# Autodesk Inventor assembly: Assembly1
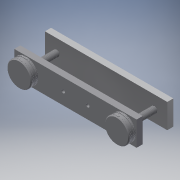
[picture p0: Inventor's stored thumbnail of the model, 180x180]
Saved by Autodesk Inventor 2019 (Build 230136000, 136)
## iProperties
Created: 2019-02-14
Part Number: Assembly1
Document SubType Name: Assembly
Designer: Delta
Author: Delta
## Documents named in this file (4)
- C:\Robotics\2018-19_CAD\lift\Assembly1.iam
- C:\Robotics\2018-19_CAD\Plate that touches lift.ipt
- C:\Robotics\2018-19_CAD\lift\Plate that doewsn't touch lander.ipt
- C:\Robotics\2018-19_CAD\lift\90210A111_LIMITED CLEARANCE SWIVEL-PAD THUMB SCREW.ipt
## Components (4 placed, 3 different names)
1. Plate that touches lift:1 — Mate:1, Mate:2
2. Plate that doewsn't touch lander:1 — Mate:3
3. 90210A111_LIMITED CLEARANCE SWIVEL-PAD THUMB SCREW:1 — Mate:2
4. 90210A111_LIMITED CLEARANCE SWIVEL-PAD THUMB SCREW:2 — Mate:1, Mate:3
## Relationships (3: Mate 3)
- Mate:1: Plate that touches lift:1 ↔ 90210A111_LIMITED CLEARANCE SWIVEL-PAD THUMB SCREW:2
- Mate:2: Plate that touches lift:1 ↔ 90210A111_LIMITED CLEARANCE SWIVEL-PAD THUMB SCREW:1
- Mate:3: Plate that doewsn't touch lander:1 ↔ 90210A111_LIMITED CLEARANCE SWIVEL-PAD THUMB SCREW:2
